# Autodesk Inventor assembly: Assembly salon y muebles
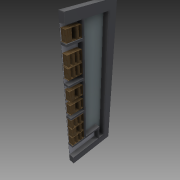
[picture p0: Inventor's stored thumbnail of the model, 180x180]
Saved by Autodesk Inventor 2015 (Build 190159000, 159)
## iProperties
Created: 2016-01-28
Part Number: Assembly salon y muebles
Document SubType Name: Assembly
Designer: 172406
Author: 172406
## Documents named in this file (4)
- H:\3d\Assembly salon y muebles.iam
- H:\3d\Assembly completo cajon gde.iam
- H:\3d\Assembly completo.iam
- H:\3d\frente salon.ipt
## Components (9 placed, 3 different names)
1. Assembly completo cajon gde:1 [sub-assembly] — Flush:2, Mate:4
2. Assembly completo:1 [sub-assembly] — Flush:1, Mate:2
3. frente salon:1 — Flush:1, Flush:2, Flush:3, Flush:4, Flush:5, Flush:6, Flush:9, Flush:10, Mate:1, Mate:2, Mate:3, Mate:4, Mate:5, Mate:6, Mate:7, Mate:8
4. Assembly completo cajon gde:2 [sub-assembly] — Flush:3, Mate:1
5. Assembly completo:2 [sub-assembly] — Flush:4, Mate:5
6. Assembly completo cajon gde:3 [sub-assembly] — Flush:5, Mate:3
7. Assembly completo:3 [sub-assembly] — Flush:6, Mate:8
8. Assembly completo cajon gde:5 [sub-assembly] — Flush:9, Mate:6
9. Assembly completo:5 [sub-assembly] — Flush:10, Mate:7
## Relationships (16: Flush 8, Mate 8)
- Flush:1: Assembly completo:1 ↔ frente salon:1
- Flush:2: Assembly completo cajon gde:1 ↔ frente salon:1
- Flush:3: frente salon:1 ↔ Assembly completo cajon gde:2
- Flush:4: frente salon:1 ↔ Assembly completo:2
- Flush:5: frente salon:1 ↔ Assembly completo cajon gde:3
- Flush:6: frente salon:1 ↔ Assembly completo:3
- Flush:9: frente salon:1 ↔ Assembly completo cajon gde:5
- Flush:10: frente salon:1 ↔ Assembly completo:5
- Mate:1: frente salon:1 ↔ Assembly completo cajon gde:2
- Mate:2: Assembly completo:1 ↔ frente salon:1
- Mate:3: frente salon:1 ↔ Assembly completo cajon gde:3
- Mate:4: Assembly completo cajon gde:1 ↔ frente salon:1
- Mate:5: frente salon:1 ↔ Assembly completo:2
- Mate:6: frente salon:1 ↔ Assembly completo cajon gde:5
- Mate:7: frente salon:1 ↔ Assembly completo:5
- Mate:8: frente salon:1 ↔ Assembly completo:3
